# Autodesk Inventor assembly: ASY mixer 2
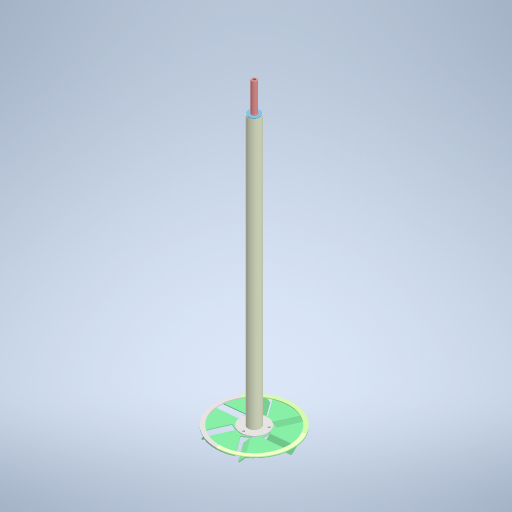
[picture p0: Inventor's stored thumbnail of the model, 512x512]
Saved by Autodesk Inventor 2024.2 (Build 282272000, 272)
## iProperties
Created: 2023-08-07
Part Number: ASY mixer 2
Document SubType Name: Assembly
Designer: admin
Author: admin
## Documents named in this file (8)
- C:\Users\pokla\Documents\Inventor\Мешалка\share\Workspaces\Workspace\станция дозирования реагента\мешалка\ASY mixer 3.iam
- C:\Users\pokla\Documents\Inventor\Мешалка\share\Workspaces\Workspace\станция дозирования реагента\мешалка\shaft 3.ipt
- C:\Users\pokla\Documents\Inventor\Мешалка\share\Workspaces\Workspace\станция дозирования реагента\мешалка\shaft 2.ipt
- C:\Users\pokla\Documents\Inventor\Мешалка\share\Workspaces\Workspace\станция дозирования реагента\мешалка\втулка.ipt
- C:\Users\pokla\Documents\Inventor\Мешалка\share\Workspaces\Workspace\станция дозирования реагента\мешалка\тарелка.ipt
- C:\Users\pokla\Documents\Inventor\Мешалка\share\Workspaces\Workspace\станция дозирования реагента\мешалка\треть-кольцо.ipt
- C:\Users\pokla\Documents\Inventor\Мешалка\share\Workspaces\Workspace\станция дозирования реагента\мешалка\платик крепежный.ipt
- C:\Users\pokla\Documents\Inventor\Мешалка\share\Workspaces\Workspace\станция дозирования реагента\мешалка\Параметры.ipt
## Components (9 placed, 7 different names)
1. shaft 3:1 — Rotational:1, Rotational:5, Mate:1, Mate:2
2. shaft 2:1 — Rotational:2
3. втулка:1 — Rotational:1, Rotational:2
4. тарелка:1 — Insert:1, Mate:1
5. платик крепежный:1 — Rotational:5, Insert:1, Mate:2
6. треть-кольцо:1 — Rigid:6, Rigid:7
7. треть-кольцо:2 — Rigid:7
8. треть-кольцо:3 — Rigid:6
9. Параметры:1
## Relationships (8: RevoluteJoint 3, WeldJoint 2, Mate 2, Insert 1)
- Rotational:1 [RevoluteJoint] (-2 mm): shaft 3:1 ↔ втулка:1
- Rotational:2 [RevoluteJoint]: shaft 2:1 ↔ втулка:1
- Rotational:5 [RevoluteJoint]: shaft 3:1 ↔ платик крепежный:1
- Rigid:6 [WeldJoint]: треть-кольцо:1 ↔ треть-кольцо:3
- Rigid:7 [WeldJoint]: треть-кольцо:1 ↔ треть-кольцо:2
- Insert:1: тарелка:1 ↔ платик крепежный:1
- Mate:1: shaft 3:1 ↔ тарелка:1
- Mate:2: shaft 3:1 ↔ платик крепежный:1
